# Autodesk Inventor assembly: mesa_aquecimento_fresamento
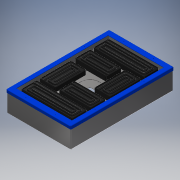
[picture p0: Inventor's stored thumbnail of the model, 180x180]
Saved by Autodesk Inventor 2018 (Build 220112000, 112)
## iProperties
Created: 2018-06-12
Part Number: mesa_aquecimento_fresamento
Material: Genérico
Document SubType Name: Assembly
Designer: Georgines
Mass: 4672.63 g
Surface Area: 8489.92 cm^2
Volume: 1688.46 cm^3
Density: 2.7674 g/cm^3
Author: Georgines
## Documents named in this file (6)
- C:\Users\Usuario\Desktop\Estação BGA\Peças 3D\mesa_aquecimento_fresamento.iam
- C:\Users\Usuario\Desktop\Estação BGA\Peças 3D\resistencia_original_2.ipt
- C:\Users\Usuario\Desktop\Estação BGA\Peças 3D\resistencia_600w.ipt
- C:\Users\Usuario\Desktop\Estação BGA\Peças 3D\mesa_suporte_resistencia_fresamento.ipt
- C:\Users\Usuario\Desktop\Estação BGA\Peças 3D\suporte_externo_fresamento.ipt
- C:\Users\Usuario\Desktop\Estação BGA\Peças 3D\tampa_mesa_resistencia_fresamento.ipt
## Components (9 placed, 5 different names)
1. resistencia_original_2:1
2. resistencia_original_2:2
3. resistencia_original_2:3
4. resistencia_original_2:4
5. resistencia_600w:1 — Coincidência:5
6. resistencia_600w:2
7. suporte_de_resistencias — Coincidência:1, Coincidência:5
8. carcaça_externa — Coincidência:1, Coincidência:2, Coincidência:3, Coincidência:4
9. tampa_superior — Coincidência:2, Coincidência:3, Coincidência:4
## Relationships (5: Mate 5)
- Coincidência:1 [Mate]: suporte_de_resistencias ↔ carcaça_externa
- Coincidência:2 [Mate]: carcaça_externa ↔ tampa_superior
- Coincidência:3 [Mate]: carcaça_externa ↔ tampa_superior
- Coincidência:4 [Mate]: carcaça_externa ↔ tampa_superior
- Coincidência:5 [Mate]: resistencia_600w:1 ↔ suporte_de_resistencias
